# Autodesk Inventor assembly: BBM Assembly
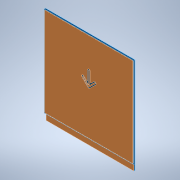
[picture p0: Inventor's stored thumbnail of the model, 180x180]
Saved by Autodesk Inventor 2022 (Build 260153000, 153)
## iProperties
Created: 2022-05-02
Part Number: BBM Assembly
Document SubType Name: Assembly
Designer: Caleb
Author: Caleb
## iProperties of the stored document board_solid.ipt
Created: 2022-05-02
Part Number: board_solid
Material: Generic
Document SubType Name: Modeling
Designer: Caleb
Density: 1 g/cm^3
Appearance: Default
Author: Caleb
## iProperties of the stored document etl_lgad_mockup_v1.iam
Created: 2022-05-02
Part Number: etl_lgad_mockup_v1
Description: FreeCAD Model
Document SubType Name: Assembly
Designer: Caleb
Authority: Unknown
Title: Open CASCADE Shape Model
Author: Author
Sending System: FreeCAD
Preprocessor: Open CASCADE STEP processor 7.5
## iProperties of the stored document etl_etroc_mockup_v1.iam
Created: 2022-04-25
Part Number: etl_etroc_mockup_v1
Description: FreeCAD Model
Document SubType Name: Assembly
Designer: Caleb
Authority: Unknown
Sending System: FreeCAD
Preprocessor: Open CASCADE STEP processor 7.5
Title: Open CASCADE Shape Model
Author: Author
## iProperties of the stored document board_solid.ipt
Created: 2022-05-02
Part Number: board_solid
Material: Generic
Document SubType Name: Modeling
Designer: Caleb
Density: 1 g/cm^3
Appearance: Default
Author: Caleb
## iProperties of the stored document copper_solid#F.Cu.ipt
Created: 2022-05-02
Part Number: copper_solid#F.Cu
Material: Generic
Document SubType Name: Modeling
Designer: Caleb
Density: 1 g/cm^3
Appearance: Default
Author: Caleb
## iProperties of the stored document copper_solid#F.Cu.ipt
Created: 2022-05-02
Part Number: copper_solid#F.Cu
Material: Generic
Document SubType Name: Modeling
Designer: Caleb
Density: 1 g/cm^3
Appearance: Default
Author: Caleb
## Documents named in this file (9)
- **C:\Users\Caleb\Desktop\nebraska-silicon-lab\Hardware\ETL\modules\throughput mockups\BBM Assembly.iam*LocalDocs*xAaaaq2daAaaaaaaaAaaaqb5oBc*board_solid.ipt
- **C:\Users\Caleb\Desktop\nebraska-silicon-lab\Hardware\ETL\modules\throughput mockups\BBM Assembly.iam*LocalDocs*xAaaaa3aaAaaaaaaaAaaaqdqrOh*etl_lgad_mockup_v1.iam
- **C:\Users\Caleb\Desktop\nebraska-silicon-lab\Hardware\ETL\modules\throughput mockups\BBM Assembly.iam*LocalDocs*xAaaaqubaAaaaaaaaAaaaaswj3c*copper_solid#F.Cu.ipt
- **C:\Users\Caleb\Desktop\nebraska-silicon-lab\Hardware\ETL\modules\throughput mockups\BBM Assembly.iam*LocalDocs*xAaaaa3aaAaaaaaaaAaaaqdqrNh*etl_etroc_mockup_v1.iam
- **C:\Users\Caleb\Desktop\nebraska-silicon-lab\Hardware\ETL\modules\throughput mockups\BBM Assembly.iam*LocalDocs*xAaaaq2daAaaaaaaaAaaaqb5oAc*board_solid.ipt
- **C:\Users\Caleb\Desktop\nebraska-silicon-lab\Hardware\ETL\modules\throughput mockups\BBM Assembly.iam*LocalDocs*xAaaaqubaAaaaaaaaAaaaaswj2c*copper_solid#F.Cu.ipt
- C:\Users\Caleb\Desktop\nebraska-silicon-lab\Hardware\ETL\modules\throughput mockups\BBM Assembly.iam
- C:\Users\Caleb\Desktop\nebraska-silicon-lab\Hardware\ETL\modules\throughput mockups\etl_etroc_mockup_v1.step
- C:\Users\Caleb\Desktop\nebraska-silicon-lab\Hardware\ETL\modules\throughput mockups\etl_lgad_mockup_v1.step
## Components (2 placed, 2 different names)
1. etl_etroc_mockup_v1:1 [sub-assembly] — Mate:1, Angle:1, Flush:1, Flush:2
2. etl_lgad_mockup_v1:1 [sub-assembly] — Mate:1, Angle:1, Flush:1, Flush:2
## Relationships (4: Flush 2, Mate 1, Angle 1)
- Mate:1: etl_etroc_mockup_v1:1 ↔ etl_lgad_mockup_v1:1
- Angle:1 (0 deg): etl_etroc_mockup_v1:1 ↔ etl_lgad_mockup_v1:1
- Flush:1 (-0.2 mm): etl_etroc_mockup_v1:1 ↔ etl_lgad_mockup_v1:1
- Flush:2 (0.2 mm): etl_etroc_mockup_v1:1 ↔ etl_lgad_mockup_v1:1
